# Autodesk Inventor assembly: yCar
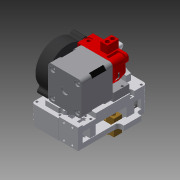
[picture p0: Inventor's stored thumbnail of the model, 180x180]
Saved by Autodesk Inventor 2013 (Build 170138000, 138)
## iProperties
Created: 2015-01-14
Part Number: yCar
Document SubType Name: Assembly
Designer: dzban
Author: dzban
## Documents named in this file (24)
- D:\PIRX\Artisan\OPENSOURCE\YCar\yCar.iam
- D:\PIRX\Artisan\OPENSOURCE\YCar\yCarBottom.ipt
- D:\PIRX\Artisan\OPENSOURCE\StockComponents\LM08UU.ipt
- D:\PIRX\Artisan\OPENSOURCE\YCar\yCarMid_a.ipt
- D:\PIRX\Artisan\OPENSOURCE\YCar\yCarMid_b.ipt
- D:\PIRX\Artisan\OPENSOURCE\YCar\yCarMid_c.ipt
- D:\PIRX\Artisan\OPENSOURCE\YCar\yCarMid_d.ipt
- D:\PIRX\Artisan\OPENSOURCE\YCar\yCarTop.ipt
- D:\PIRX\Artisan\OPENSOURCE\YCar\yCarTopper.ipt
- D:\PIRX\Artisan\OPENSOURCE\YCar\yCarWireHolder.ipt
- D:\PIRX\Artisan\OPENSOURCE\YCar\yCarBeltTensionerHolder.ipt
- D:\PIRX\Artisan\OPENSOURCE\YCar\yCarBeltTensioner.ipt
- D:\PIRX\Artisan\OPENSOURCE\YCar\dysza_abs2.ipt
- D:\PIRX\Artisan\OPENSOURCE\YCar\exTeflonTube.ipt
- D:\PIRX\Artisan\OPENSOURCE\YCar\exAluBase.ipt
- D:\PIRX\Artisan\OPENSOURCE\YCar\exBolt.ipt
- D:\PIRX\Artisan\OPENSOURCE\YCar\exHeaterBlock.ipt
- D:\PIRX\Artisan\OPENSOURCE\YCar\exNozzle.ipt
- D:\PIRX\Artisan\OPENSOURCE\YCar\exStSteelTube.ipt
- D:\PIRX\Artisan\OPENSOURCE\StockComponents\NEMA17Stepper.ipt
- D:\PIRX\Artisan\OPENSOURCE\StockComponents\blowerFan50x15.ipt
- D:\PIRX\Artisan\OPENSOURCE\YCar\exTop.ipt
- D:\PIRX\Artisan\OPENSOURCE\YCar\exLever.ipt
- D:\PIRX\Artisan\OPENSOURCE\StockComponents\695ZZ_bearing.ipt
## Components (31 placed, 23 different names)
1. yCarBottom:1 — Mate:1, Mate:2, Mate:3, Tangent:1, Tangent:2, Tangent:3, Tangent:4, Tangent:5, Tangent:6, Insert:1, Insert:3, Insert:5, Insert:7, Insert:9, Insert:11, Insert:13, Insert:14, Insert:17, Insert:19, Flush:1, Flush:2, Mate:8, Insert:25, Insert:26
2. LM08UU:1 — Mate:3, Tangent:2, Tangent:5
3. LM08UU:2 — Mate:2, Tangent:3, Tangent:6
4. LM08UU:3 — Mate:1, Tangent:1, Tangent:4
5. yCarMid_a:1 — Insert:1, Insert:2, Insert:11, Insert:12
6. yCarMid_a:2 — Insert:2, Insert:12, Insert:22
7. yCarMid_b:1 — Insert:3, Insert:4, Insert:9, Insert:10
8. yCarMid_b:2 — Insert:4, Insert:10
9. yCarMid_b:3 — Insert:5, Insert:6, Insert:7, Insert:8
10. yCarMid_b:4 — Insert:6, Insert:8, Insert:21
11. yCarMid_c:1 — Insert:15, Insert:16
12. yCarMid_c:2 — Insert:13, Insert:14, Insert:15, Insert:16
13. yCarMid_d:1 — Insert:18, Insert:20
14. yCarMid_d:2 — Insert:17, Insert:18, Insert:19, Insert:20
15. yCarTop:1 — Insert:21, Insert:22, Insert:23, Insert:24, Mate:6, Mate:7, Mate:10, Mate:11
16. yCarTopper:1 — Mate:4, Mate:5, Tangent:7, Insert:23, Insert:24, Insert:31, Angle:1, Mate:9
17. yCarWireHolder:1 — Mate:4, Mate:5, Tangent:7
18. yCarBeltTensionerHolder:1 — Mate:7, Flush:2, Mate:8
19. yCarBeltTensioner:1 — Flush:1, Mate:6
20. dysza_abs2:1 — Insert:25, Insert:26
21. exTeflonTube:1 — Insert:29
22. exAluBase:1 — Insert:27, Insert:31, Angle:1, Insert:32, Insert:33
23. exBolt:1 — Insert:34
24. exHeaterBlock:1 — Insert:28, Insert:30
25. exNozzle:1 — Insert:28
26. exStSteelTube:1 — Insert:27, Insert:29, Insert:30
27. NEMA17Stepper:1 — Insert:32, Insert:33, Insert:34, Insert:35, Insert:36
28. blowerFan50x15:1 — Mate:9, Mate:10, Mate:11
29. exTop:1 — Insert:35, Insert:36, Insert:37
30. exLever:1 — Insert:37, Insert:38
31. 695ZZ_bearing:1 — Insert:38
## Relationships (59: Insert 38, Mate 11, Tangent 7, Flush 2, Angle 1)
- Mate:1: yCarBottom:1 ↔ LM08UU:3
- Mate:2: yCarBottom:1 ↔ LM08UU:2
- Mate:3: yCarBottom:1 ↔ LM08UU:1
- Tangent:1: yCarBottom:1 ↔ LM08UU:3
- Tangent:2: yCarBottom:1 ↔ LM08UU:1
- Tangent:3: yCarBottom:1 ↔ LM08UU:2
- Tangent:4: yCarBottom:1 ↔ LM08UU:3
- Tangent:5: yCarBottom:1 ↔ LM08UU:1
- Tangent:6: yCarBottom:1 ↔ LM08UU:2
- Insert:1: yCarBottom:1 ↔ yCarMid_a:1
- Insert:2: yCarMid_a:1 ↔ yCarMid_a:2
- Insert:3: yCarBottom:1 ↔ yCarMid_b:1
- Insert:4: yCarMid_b:1 ↔ yCarMid_b:2
- Insert:5: yCarBottom:1 ↔ yCarMid_b:3
- Insert:6: yCarMid_b:3 ↔ yCarMid_b:4
- Insert:7: yCarBottom:1 ↔ yCarMid_b:3
- Insert:8: yCarMid_b:3 ↔ yCarMid_b:4
- Insert:9: yCarBottom:1 ↔ yCarMid_b:1
- Insert:10: yCarMid_b:1 ↔ yCarMid_b:2
- Insert:11: yCarBottom:1 ↔ yCarMid_a:1
- Insert:12: yCarMid_a:1 ↔ yCarMid_a:2
- Insert:13: yCarBottom:1 ↔ yCarMid_c:2
- Insert:14: yCarBottom:1 ↔ yCarMid_c:2
- Insert:15: yCarMid_c:1 ↔ yCarMid_c:2
- Insert:16: yCarMid_c:1 ↔ yCarMid_c:2
- Insert:17: yCarBottom:1 ↔ yCarMid_d:2
- Insert:18: yCarMid_d:1 ↔ yCarMid_d:2
- Insert:19: yCarBottom:1 ↔ yCarMid_d:2
- Insert:20: yCarMid_d:1 ↔ yCarMid_d:2
- Insert:21: yCarMid_b:4 ↔ yCarTop:1
- Mate:4: yCarTopper:1 ↔ yCarWireHolder:1
- Mate:5: yCarTopper:1 ↔ yCarWireHolder:1
- Tangent:7: yCarTopper:1 ↔ yCarWireHolder:1
- Insert:22: yCarMid_a:2 ↔ yCarTop:1
- Insert:23: yCarTop:1 ↔ yCarTopper:1
- Insert:24: yCarTop:1 ↔ yCarTopper:1
- Flush:1: yCarBottom:1 ↔ yCarBeltTensioner:1
- Mate:6: yCarTop:1 ↔ yCarBeltTensioner:1
- Mate:7: yCarTop:1 ↔ yCarBeltTensionerHolder:1
- Flush:2: yCarBottom:1 ↔ yCarBeltTensionerHolder:1
- Mate:8: yCarBottom:1 ↔ yCarBeltTensionerHolder:1
- Insert:25: yCarBottom:1 ↔ dysza_abs2:1
- Insert:26: yCarBottom:1 ↔ dysza_abs2:1
- Insert:27 (-6 mm): exAluBase:1 ↔ exStSteelTube:1
- Insert:28 (-6 mm): exHeaterBlock:1 ↔ exNozzle:1
- Insert:29 (-42 mm): exTeflonTube:1 ↔ exStSteelTube:1
- Insert:30 (-4 mm): exHeaterBlock:1 ↔ exStSteelTube:1
- Insert:31: yCarTopper:1 ↔ exAluBase:1
- Angle:1 (0 deg): yCarTopper:1 ↔ exAluBase:1
- Insert:32: exAluBase:1 ↔ NEMA17Stepper:1
- Insert:33: exAluBase:1 ↔ NEMA17Stepper:1
- Insert:34: exBolt:1 ↔ NEMA17Stepper:1
- Mate:9: yCarTopper:1 ↔ blowerFan50x15:1
- Mate:10: yCarTop:1 ↔ blowerFan50x15:1
- Mate:11 (-3 mm): yCarTop:1 ↔ blowerFan50x15:1
- Insert:35: NEMA17Stepper:1 ↔ exTop:1
- Insert:36: NEMA17Stepper:1 ↔ exTop:1
- Insert:37 (1 mm): exTop:1 ↔ exLever:1
- Insert:38: exLever:1 ↔ 695ZZ_bearing:1
